# Autodesk Inventor assembly: Motor Mount HSI
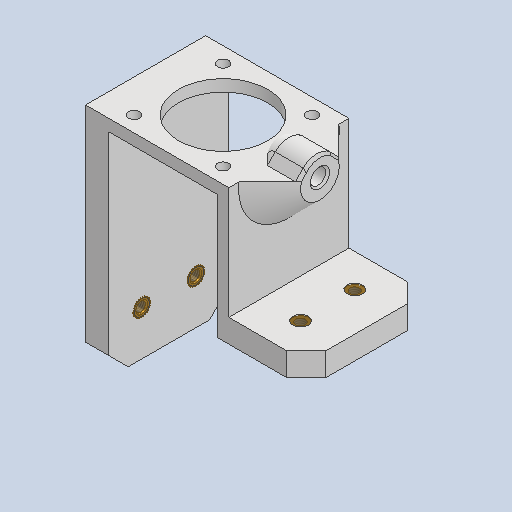
[picture p0: Inventor's stored thumbnail of the model, 512x512]
Saved by Autodesk Inventor 2022 (Build 260153000, 153)
## iProperties
Created: 2022-06-07
Part Number: Motor Mount HSI
Document SubType Name: Assembly
Designer: Nick
Author: Nick
## Documents named in this file (3)
- Y:\Projects\Mini_Sand_Table\Motor Mount HSI.iam
- Y:\Projects\Mini_Sand_Table\Motor Mount.ipt
- Y:\Projects\Mini_Sand_Table\M3 Heat Set Inserts.ipt
## Components (5 placed, 2 different names)
1. Motor Mount:1 — Insert:1, Insert:2, Insert:3, Insert:4
2. M3 Heat Set Inserts:1 — Insert:1
3. M3 Heat Set Inserts:2 — Insert:2
4. M3 Heat Set Inserts:3 — Insert:3
5. M3 Heat Set Inserts:4 — Insert:4
## Relationships (4: Insert 4)
- Insert:1: Motor Mount:1 ↔ M3 Heat Set Inserts:1
- Insert:2: Motor Mount:1 ↔ M3 Heat Set Inserts:2
- Insert:3: Motor Mount:1 ↔ M3 Heat Set Inserts:3
- Insert:4: Motor Mount:1 ↔ M3 Heat Set Inserts:4
